# Autodesk Inventor assembly: Montagem Ferramental
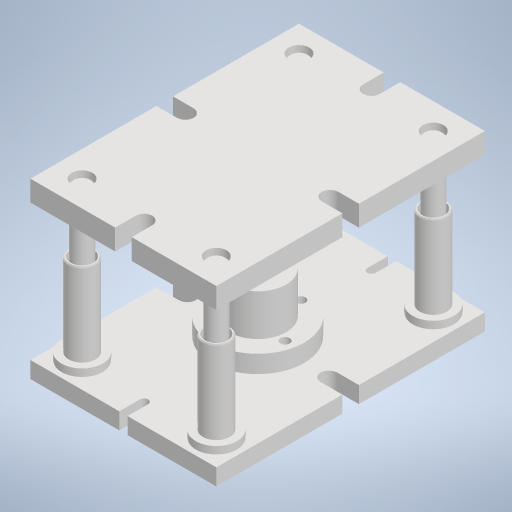
[picture p0: Inventor's stored thumbnail of the model, 512x512]
Saved by Autodesk Inventor 2023.2 (Build 272271000, 271)
## iProperties
Created: 2022-12-17
Part Number: Montagem Ferramental
Document SubType Name: Assembly
Designer: Felipe Coquito
Checked By: Felipe Mello
Engr Approved By: Felipe Mello
Description: Ferramental 045
Mass: 2197.1 g
Surface Area: 3919.87 cm^2
Volume: 2197.1 cm^3
Density: 1 g/cm^3
Author: coqui
## Documents named in this file (7)
- D:\Felipe Coquito\OneDrive\Documents\Inventor\Inventor - curso\Montagem\Montagem Ferramental.iam
- D:\Felipe Coquito\OneDrive\Documents\Inventor\Inventor - curso\Ferramental\Base inferior da ferramenta.ipt
- D:\Felipe Coquito\OneDrive\Documents\Inventor\Inventor - curso\Ferramental\Coluna do Ferramental.ipt
- D:\Felipe Coquito\OneDrive\Documents\Inventor\Inventor - curso\Ferramental\Matriz inferior do Ferramental.ipt
- D:\Felipe Coquito\OneDrive\Documents\Inventor\Inventor - curso\Ferramental\Bucha do Ferramental.ipt
- D:\Felipe Coquito\OneDrive\Documents\Inventor\Inventor - curso\Ferramental\Base superior da ferramenta.ipt
- D:\Felipe Coquito\OneDrive\Documents\Inventor\Inventor - curso\Ferramental\Matriz superior do Ferramental.ipt
## Components (12 placed, 6 different names)
1. Base inferior da ferramenta:1 — Mate:1, Mate:2, Mate:3, Mate:4, Mate:5, Mate:6, Mate:7, Mate:8, Mate:9, Mate:10, Mate:11, Angle:1, Angle:2
2. Coluna do Ferramental:1 — Mate:1, Mate:2, Mate:16, Mate:17
3. Coluna do Ferramental:2 — Mate:3, Mate:4, Mate:14, Mate:15
4. Coluna do Ferramental:3 — Mate:5, Mate:6, Mate:12, Mate:13
5. Coluna do Ferramental:4 — Mate:7, Mate:8, Mate:18, Mate:19
6. Matriz inferior do Ferramental:1 — Mate:9, Mate:10, Mate:11, Mate:26
7. Bucha do Ferramental:1 — Mate:12, Mate:13, Mate:23, Flush:3
8. Bucha do Ferramental:2 — Mate:14, Mate:15, Mate:22, Flush:4
9. Bucha do Ferramental:3 — Mate:16, Mate:17, Mate:21, Flush:1
10. Bucha do Ferramental:4 — Mate:18, Mate:19, Mate:20, Mate:24, Flush:2
11. Base superior da ferramenta:1 — Mate:20, Mate:21, Mate:22, Mate:23, Mate:24, Mate:25, Flush:1, Flush:2, Flush:3, Flush:4
12. Matriz superior do Ferramental:1 — Mate:25, Mate:26
## Relationships (32: Mate 26, Flush 4, Angle 2)
- Mate:1: Base inferior da ferramenta:1 ↔ Coluna do Ferramental:1
- Mate:2: Base inferior da ferramenta:1 ↔ Coluna do Ferramental:1
- Mate:3: Base inferior da ferramenta:1 ↔ Coluna do Ferramental:2
- Mate:4: Base inferior da ferramenta:1 ↔ Coluna do Ferramental:2
- Mate:5: Base inferior da ferramenta:1 ↔ Coluna do Ferramental:3
- Mate:6: Base inferior da ferramenta:1 ↔ Coluna do Ferramental:3
- Mate:7: Base inferior da ferramenta:1 ↔ Coluna do Ferramental:4
- Mate:8: Base inferior da ferramenta:1 ↔ Coluna do Ferramental:4
- Mate:9: Base inferior da ferramenta:1 ↔ Matriz inferior do Ferramental:1
- Mate:10: Base inferior da ferramenta:1 ↔ Matriz inferior do Ferramental:1
- Mate:11: Base inferior da ferramenta:1 ↔ Matriz inferior do Ferramental:1
- Mate:12: Coluna do Ferramental:3 ↔ Bucha do Ferramental:1
- Mate:13: Coluna do Ferramental:3 ↔ Bucha do Ferramental:1
- Mate:14: Coluna do Ferramental:2 ↔ Bucha do Ferramental:2
- Mate:15: Coluna do Ferramental:2 ↔ Bucha do Ferramental:2
- Mate:16: Coluna do Ferramental:1 ↔ Bucha do Ferramental:3
- Mate:17: Coluna do Ferramental:1 ↔ Bucha do Ferramental:3
- Mate:18: Coluna do Ferramental:4 ↔ Bucha do Ferramental:4
- Mate:19: Coluna do Ferramental:4 ↔ Bucha do Ferramental:4
- Mate:20: Bucha do Ferramental:4 ↔ Base superior da ferramenta:1
- Mate:21: Bucha do Ferramental:3 ↔ Base superior da ferramenta:1
- Mate:22: Bucha do Ferramental:2 ↔ Base superior da ferramenta:1
- Mate:23: Bucha do Ferramental:1 ↔ Base superior da ferramenta:1
- Mate:24: Bucha do Ferramental:4 ↔ Base superior da ferramenta:1
- Mate:25: Base superior da ferramenta:1 ↔ Matriz superior do Ferramental:1
- Mate:26: Matriz inferior do Ferramental:1 ↔ Matriz superior do Ferramental:1
- Flush:1: Bucha do Ferramental:3 ↔ Base superior da ferramenta:1
- Flush:2: Bucha do Ferramental:4 ↔ Base superior da ferramenta:1
- Flush:3: Bucha do Ferramental:1 ↔ Base superior da ferramenta:1
- Flush:4: Bucha do Ferramental:2 ↔ Base superior da ferramenta:1
- Angle:1 (0 deg): Base inferior da ferramenta:1
- Angle:2 (0 deg): Base inferior da ferramenta:1
